# Autodesk Inventor assembly: Senior Project Assembly
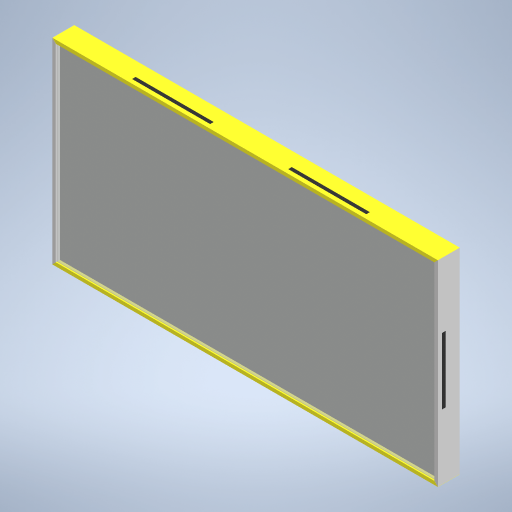
[picture p0: Inventor's stored thumbnail of the model, 512x512]
Saved by Autodesk Inventor 2024 (Build 280153000, 153)
## iProperties
Created: 2024-02-22
Part Number: Senior Project Assembly
Document SubType Name: Assembly
Designer: flynf
Author: flynf
## Documents named in this file (5)
- C:\Users\flynf\Documents\Senior Project Assembly.iam
- C:\Users\flynf\Documents\Final Product backplate.ipt
- C:\Users\flynf\Documents\Frame Side(Long).ipt
- C:\Users\flynf\Documents\Frame Side(Short).ipt
- C:\Users\flynf\Documents\Clear Panel.ipt
## Components (6 placed, 4 different names)
1. Final Product backplate:1 — Flush:1, Mate:3, Mate:4, Flush:2, Mate:5, Mate:6, Flush:3, Mate:8, Mate:9, Flush:4, Mate:10, Mate:11
2. Clear Panel:1 — Mate:1, Mate:2, Mate:7
3. Frame Side(Long):1 — Mate:1, Mate:2, Flush:1, Mate:3, Mate:4
4. Frame Side(Short):1 — Flush:2, Mate:5, Mate:6, Mate:7
5. Frame Side(Short):2 — Flush:3, Mate:8, Mate:9
6. Frame Side(Long):2 — Flush:4, Mate:10, Mate:11
## Relationships (15: Mate 11, Flush 4)
- Mate:1: Clear Panel:1 ↔ Frame Side(Long):1
- Mate:2: Clear Panel:1 ↔ Frame Side(Long):1
- Flush:1: Final Product backplate:1 ↔ Frame Side(Long):1
- Mate:3: Final Product backplate:1 ↔ Frame Side(Long):1
- Mate:4: Final Product backplate:1 ↔ Frame Side(Long):1
- Flush:2: Final Product backplate:1 ↔ Frame Side(Short):1
- Mate:5: Final Product backplate:1 ↔ Frame Side(Short):1
- Mate:6: Final Product backplate:1 ↔ Frame Side(Short):1
- Mate:7: Clear Panel:1 ↔ Frame Side(Short):1
- Flush:3: Final Product backplate:1 ↔ Frame Side(Short):2
- Mate:8: Final Product backplate:1 ↔ Frame Side(Short):2
- Mate:9: Final Product backplate:1 ↔ Frame Side(Short):2
- Flush:4: Final Product backplate:1 ↔ Frame Side(Long):2
- Mate:10: Final Product backplate:1 ↔ Frame Side(Long):2
- Mate:11: Final Product backplate:1 ↔ Frame Side(Long):2
